# Autodesk Inventor assembly: FrameV3
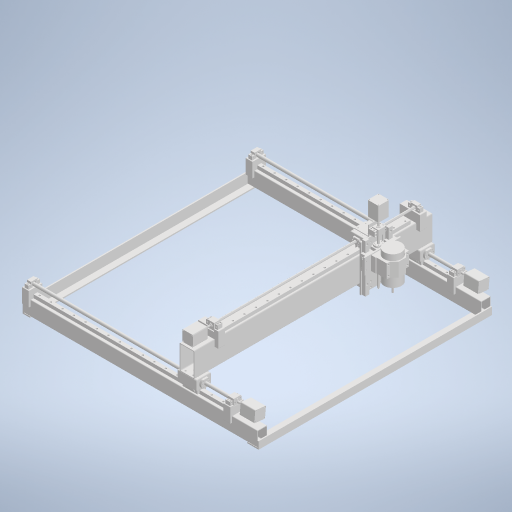
[picture p0: Inventor's stored thumbnail of the model, 512x512]
Saved by Autodesk Inventor 2023 (Build 270158000, 158)
## iProperties
Created: 2022-05-03
Part Number: FrameV3
Document SubType Name: Assembly
Designer: plebbb
Author: plebbb
## Documents named in this file (15)
- D:\Users\plebbb\Desktop\CNC_Project\FrameV3.iam
- D:\Users\plebbb\Desktop\CNC_Project\Ballscrew_Assembly.iam
- D:\Users\plebbb\Desktop\CNC_Project\X_GANTRY.iam
- D:\Users\plebbb\Desktop\CNC_Project\Steel_L_Bracket.ipt
- D:\Users\plebbb\Desktop\CNC_Project\Spindle.ipt
- D:\Users\plebbb\Desktop\CNC_Project\Spindle_Holder.ipt
- D:\Users\plebbb\Desktop\CNC_Project\Z_PLATE.iam
- D:\Users\plebbb\Desktop\CNC_Project\Y_GANTRY.iam
- D:\Users\plebbb\Desktop\CNC_Project\Z_GANTRY.iam
- D:\Users\plebbb\Desktop\CNC_Project\FrameV3\AIP\FEA\dyol7vh0g.fins
- D:\Users\plebbb\Desktop\CNC_Project\FrameV3\AIP\FEA\dyol7vh0g.fsat
- D:\Users\plebbb\Desktop\CNC_Project\FrameV3\AIP\FEA\dyol7vh0g.ftes
- D:\Users\plebbb\Desktop\CNC_Project\FrameV3\AIP\FEA\dyol7vh0g.fwiz
- D:\Users\plebbb\Desktop\CNC_Project\FrameV3\AIP\FEA\dyol7vheo.fmsh
- D:\Users\plebbb\Desktop\CNC_Project\FrameV3\AIP\FEA\dyol7vhep.fres
## Components (11 placed, 8 different names)
1. Ballscrew_Assembly:1 [sub-assembly] — Mate:93
2. X_GANTRY:1 [sub-assembly] — Mate:30, Mate:31, Flush:4, Mate:38, Flush:9, Mate:40, Flush:49
3. X_GANTRY:2 [sub-assembly] — Mate:25, Mate:26, Mate:27, Mate:28, Mate:29, Mate:34, Mate:37, Flush:6, Mate:39, Flush:8
4. Ballscrew_Assembly:2 [sub-assembly] — Mate:25, Mate:26, Mate:27, Mate:28, Mate:29, Mate:94, Mate:95
5. Steel_L_Bracket:1 — Mate:30, Mate:31, Flush:4, Mate:34, Mate:37, Flush:6, Flush:42, Mate:42, Mate:69
6. Steel_L_Bracket:3 — Mate:38, Mate:39, Flush:8, Flush:9, Mate:40
7. Spindle:1 — Mate:70, Flush:43, Flush:49
8. Spindle_Holder:1 — Mate:70, Flush:43
9. Z_PLATE:1 [sub-assembly] — Mate:97, Mate:98, Mate:99
10. Y_GANTRY:1 [sub-assembly] — Mate:93, Mate:94, Mate:95, Mate:96, Angle:1
11. Z_GANTRY:1 [sub-assembly] — Mate:96, Angle:1, Mate:97, Mate:98, Mate:99
## Relationships (41: Mate 31, Flush 9, Angle 1)
- [Mate]: Ballscrew_Assembly:1 ↔ X_GANTRY:1
- [Mate]: Ballscrew_Assembly:1 ↔ X_GANTRY:1
- [Flush]: Ballscrew_Assembly:1 ↔ X_GANTRY:1
- [Flush]: Ballscrew_Assembly:1 ↔ X_GANTRY:1
- [Mate]: Ballscrew_Assembly:1 ↔ X_GANTRY:1
- [Mate]: Ballscrew_Assembly:1 ↔ X_GANTRY:1
- [Mate]: Ballscrew_Assembly:1 ↔ X_GANTRY:1
- [Mate]: Ballscrew_Assembly:1 ↔ X_GANTRY:1
- Mate:25: X_GANTRY:2 ↔ Ballscrew_Assembly:2
- Mate:26: X_GANTRY:2 ↔ Ballscrew_Assembly:2
- Mate:27: X_GANTRY:2 ↔ Ballscrew_Assembly:2
- Mate:28: X_GANTRY:2 ↔ Ballscrew_Assembly:2
- Mate:29: X_GANTRY:2 ↔ Ballscrew_Assembly:2
- Mate:30: X_GANTRY:1 ↔ Steel_L_Bracket:1
- Mate:31: X_GANTRY:1 ↔ Steel_L_Bracket:1
- Flush:4: X_GANTRY:1 ↔ Steel_L_Bracket:1
- Mate:34: X_GANTRY:2 ↔ Steel_L_Bracket:1
- Mate:37: X_GANTRY:2 ↔ Steel_L_Bracket:1
- Flush:6: X_GANTRY:2 ↔ Steel_L_Bracket:1
- Mate:38: X_GANTRY:1 ↔ Steel_L_Bracket:3
- Mate:39: X_GANTRY:2 ↔ Steel_L_Bracket:3
- Flush:8: X_GANTRY:2 ↔ Steel_L_Bracket:3
- Flush:9: X_GANTRY:1 ↔ Steel_L_Bracket:3
- Mate:40: X_GANTRY:1 ↔ Steel_L_Bracket:3
- Flush:42: Steel_L_Bracket:1
- Mate:42: Steel_L_Bracket:1
- Mate:69: Steel_L_Bracket:1
- Mate:70: Spindle:1 ↔ Spindle_Holder:1
- Flush:43 (50 mm): Spindle:1 ↔ Spindle_Holder:1
- [Mate]: Spindle_Holder:1 ↔ Z_PLATE:1
- [Mate]: Spindle_Holder:1 ↔ Z_PLATE:1
- [Mate]: Spindle_Holder:1 ↔ Z_PLATE:1
- Flush:49: X_GANTRY:1 ↔ Spindle:1
- Mate:93: Ballscrew_Assembly:1 ↔ Y_GANTRY:1
- Mate:94: Ballscrew_Assembly:2 ↔ Y_GANTRY:1
- Mate:95: Ballscrew_Assembly:2 ↔ Y_GANTRY:1
- Mate:96: Y_GANTRY:1 ↔ Z_GANTRY:1
- Angle:1 (180 deg): Y_GANTRY:1 ↔ Z_GANTRY:1
- Mate:97: Z_PLATE:1 ↔ Z_GANTRY:1
- Mate:98: Z_PLATE:1 ↔ Z_GANTRY:1
- Mate:99: Z_PLATE:1 ↔ Z_GANTRY:1
## Named parameters: sa_0 = 100000
note: some values were not read from the file. Shown as the stored number, unit unknown: "sa_0".
